# Autodesk Inventor assembly: CameraAssembly
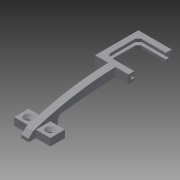
[picture p0: Inventor's stored thumbnail of the model, 180x180]
Saved by Autodesk Inventor 2015 (Build 190159000, 159)
## iProperties
Created: 2015-11-25
Part Number: CameraAssembly
Document SubType Name: Assembly
Designer: Lauszus
Author: Lauszus
## Documents named in this file (4)
- C:\Users\Lauszus\Dropbox\DTU\7. semester\Image Analysis with Microcomputer - 30330\Lab exercises\ObjectTracking\3DModel\CameraAssembly.iam
- C:\Users\Lauszus\Dropbox\DTU\7. semester\Image Analysis with Microcomputer - 30330\Lab exercises\ObjectTracking\3DModel\CameraArmMount.ipt
- C:\Users\Lauszus\Dropbox\DTU\7. semester\Image Analysis with Microcomputer - 30330\Lab exercises\ObjectTracking\3DModel\CameraArm.ipt
- C:\Users\Lauszus\Dropbox\DTU\7. semester\Image Analysis with Microcomputer - 30330\Lab exercises\ObjectTracking\3DModel\CameraHolder.ipt
## Components (3 placed, 3 different names)
1. CameraArmMount:1 — Mate:1, Mate:2, Mate:3, Flush:2
2. CameraArm:1 — Mate:1, Mate:2, Mate:3, Mate:4, Flush:1
3. CameraHolder:1 — Mate:4, Flush:1, Flush:2
## Relationships (6: Mate 4, Flush 2)
- Mate:1: CameraArmMount:1 ↔ CameraArm:1
- Mate:2: CameraArmMount:1 ↔ CameraArm:1
- Mate:3: CameraArmMount:1 ↔ CameraArm:1
- Mate:4: CameraArm:1 ↔ CameraHolder:1
- Flush:1 (9 mm): CameraArm:1 ↔ CameraHolder:1
- Flush:2 (10 mm): CameraArmMount:1 ↔ CameraHolder:1
